# Autodesk Inventor assembly: Right Leg Assembly
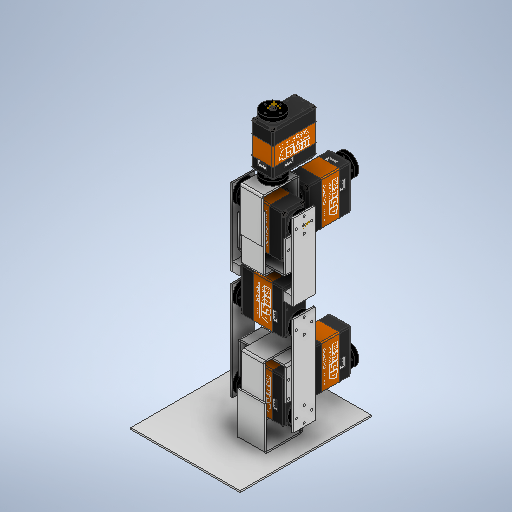
[picture p0: Inventor's stored thumbnail of the model, 512x512]
Saved by Autodesk Inventor 2025.2 (Build 292293000, 293)
## iProperties
Created: 2025-05-04
Part Number: Right Leg Assembly
Document SubType Name: Assembly
Designer: User
Author: User
## Documents named in this file (10)
- C:\Users\User\Documents\The Maverick's Files\College 3-3\로보인 프로젝트\Leg Parts\Right Leg Assembly.iam
- C:\Users\User\Documents\The Maverick's Files\College 3-3\로보인 프로젝트\Leg Parts\axis_12_bottom_frame(bottom).ipt
- C:\Users\User\Documents\The Maverick's Files\College 3-3\로보인 프로젝트\Leg Parts\axis_12_bottom_frame(top).ipt
- C:\Users\User\Documents\The Maverick's Files\College 3-3\로보인 프로젝트\RHp_hardware_example\Part\HTD-45H, Horn\HTD-45H Assembly.iam
- C:\Users\User\Documents\The Maverick's Files\College 3-3\로보인 프로젝트\Leg Parts\axis_10_11-connector_frame.ipt
- C:\Users\User\Documents\The Maverick's Files\College 3-3\로보인 프로젝트\Leg Parts\axis_9_bottom_frame.ipt
- C:\Users\User\Documents\The Maverick's Files\College 3-3\로보인 프로젝트\Leg Parts\axis_10_top_frame.ipt
- C:\Users\User\Documents\The Maverick's Files\College 3-3\로보인 프로젝트\Leg Parts\axis_8_10_connector_frame.ipt
- C:\Users\User\Documents\The Maverick's Files\College 3-3\로보인 프로젝트\Leg Parts\axis_7_top_frame.ipt
- C:\Users\User\Documents\The Maverick's Files\College 3-3\로보인 프로젝트\Leg Parts\3D_printed_part.ipt
## Components (19 placed, 9 different names)
1. axis_12_bottom_frame(bottom):1 — Mate:1, Mate:2, Mate:3, Mate:4, Mate:5, Mate:6, Mate:9, Mate:11, Mate:13
2. axis_12_bottom_frame(top):1 — Mate:4, Mate:5, Mate:6, Mate:10, Mate:12, Flush:1, Mate:14, Mate:15, Mate:16, Mate:22, Mate:25, Flush:5
3. HTD-45H Assembly:1 [sub-assembly] — Mate:12, Flush:1, Mate:13
4. HTD-45H Assembly:2 [sub-assembly] — Mate:9, Mate:10, Mate:11, Mate:20, Mate:21, Mate:23, Mate:24, Mate:26, Flush:2
5. HTD-45H Assembly:3 [sub-assembly] — Mate:27, Mate:28, Flush:2, Mate:29, Mate:30, Mate:31, Mate:32, Mate:35, Mate:37
6. HTD-45H Assembly:4 [sub-assembly] — Mate:33, Mate:34, Mate:35, Mate:36, Mate:40, Flush:9, Mate:44, Flush:10
7. HTD-45H Assembly:5 [sub-assembly] — Mate:41, Mate:42, Flush:9
8. HTD-45H Assembly:6 [sub-assembly] — Flush:5, Mate:36, Mate:37, Mate:38, Flush:6, Flush:7
9. axis_10_11-connector_frame:1 — Mate:23, Mate:24, Mate:25, Mate:27, Mate:28, Flush:4
10. axis_10_11-connector_frame:2 — Mate:20, Mate:21, Mate:22, Flush:3
11. axis_9_bottom_frame:1 — Mate:14, Mate:15, Mate:16, Mate:17, Mate:19
12. axis_10_top_frame:1 — Mate:17, Mate:19, Mate:26
13. axis_8_10_connector_frame:1 — Mate:29, Mate:30, Flush:3, Flush:11, Mate:45, Flush:12
14. axis_8_10_connector_frame:2 — Mate:31, Mate:32, Flush:4, Mate:33, Mate:34, Flush:13, Mate:46, Flush:14
15. axis_7_top_frame:1 — Mate:38, Flush:6, Flush:7, Mate:39, Flush:8
16. axis_9_bottom_frame:2 — Mate:39, Flush:8, Mate:40, Mate:41, Mate:42, Mate:43
17. axis_10_top_frame:2 — Mate:43, Mate:44, Flush:10
18. 3D_printed_part:1 — Flush:11, Mate:45, Flush:12
19. 3D_printed_part:2 — Flush:13, Mate:46, Flush:14
## Relationships (57: Mate 43, Flush 14)
- Mate:1: axis_12_bottom_frame(bottom):1
- Mate:2: axis_12_bottom_frame(bottom):1
- Mate:3: axis_12_bottom_frame(bottom):1
- Mate:4: axis_12_bottom_frame(bottom):1 ↔ axis_12_bottom_frame(top):1
- Mate:5 (-20 mm): axis_12_bottom_frame(bottom):1 ↔ axis_12_bottom_frame(top):1
- Mate:6 (-20 mm): axis_12_bottom_frame(bottom):1 ↔ axis_12_bottom_frame(top):1
- Mate:9: axis_12_bottom_frame(bottom):1 ↔ HTD-45H Assembly:2
- Mate:10 (-20 mm): axis_12_bottom_frame(top):1 ↔ HTD-45H Assembly:2
- Mate:11 (-30 mm): axis_12_bottom_frame(bottom):1 ↔ HTD-45H Assembly:2
- Mate:12: axis_12_bottom_frame(top):1 ↔ HTD-45H Assembly:1
- Flush:1: axis_12_bottom_frame(top):1 ↔ HTD-45H Assembly:1
- Mate:13 (-30 mm): axis_12_bottom_frame(bottom):1 ↔ HTD-45H Assembly:1
- Mate:14: axis_12_bottom_frame(top):1 ↔ axis_9_bottom_frame:1
- Mate:15: axis_12_bottom_frame(top):1 ↔ axis_9_bottom_frame:1
- Mate:16 (71.5 mm): axis_12_bottom_frame(top):1 ↔ axis_9_bottom_frame:1
- Mate:17: axis_9_bottom_frame:1 ↔ axis_10_top_frame:1
- Mate:19 (1.5 mm): axis_9_bottom_frame:1 ↔ axis_10_top_frame:1
- Mate:20: HTD-45H Assembly:2 ↔ axis_10_11-connector_frame:2
- Mate:21: HTD-45H Assembly:2 ↔ axis_10_11-connector_frame:2
- Mate:22 (20 mm): axis_12_bottom_frame(top):1 ↔ axis_10_11-connector_frame:2
- Mate:23: HTD-45H Assembly:2 ↔ axis_10_11-connector_frame:1
- Mate:24: HTD-45H Assembly:2 ↔ axis_10_11-connector_frame:1
- Mate:25 (20 mm): axis_12_bottom_frame(top):1 ↔ axis_10_11-connector_frame:1
- Mate:26: HTD-45H Assembly:2 ↔ axis_10_top_frame:1
- Mate:27: HTD-45H Assembly:3 ↔ axis_10_11-connector_frame:1
- Mate:28: HTD-45H Assembly:3 ↔ axis_10_11-connector_frame:1
- Flush:2 (-70 mm): HTD-45H Assembly:2 ↔ HTD-45H Assembly:3
- Mate:29 (-10 mm): HTD-45H Assembly:3 ↔ axis_8_10_connector_frame:1
- Mate:30: HTD-45H Assembly:3 ↔ axis_8_10_connector_frame:1
- Flush:3: axis_10_11-connector_frame:2 ↔ axis_8_10_connector_frame:1
- Mate:31 (-10 mm): HTD-45H Assembly:3 ↔ axis_8_10_connector_frame:2
- Mate:32: HTD-45H Assembly:3 ↔ axis_8_10_connector_frame:2
- Flush:4: axis_10_11-connector_frame:1 ↔ axis_8_10_connector_frame:2
- Mate:33: HTD-45H Assembly:4 ↔ axis_8_10_connector_frame:2
- Mate:34: HTD-45H Assembly:4 ↔ axis_8_10_connector_frame:2
- Mate:35 (80 mm): HTD-45H Assembly:3 ↔ HTD-45H Assembly:4
- Flush:5: axis_12_bottom_frame(top):1 ↔ HTD-45H Assembly:6
- Mate:36: HTD-45H Assembly:4 ↔ HTD-45H Assembly:6
- Mate:37 (80 mm): HTD-45H Assembly:3 ↔ HTD-45H Assembly:6
- Mate:38: HTD-45H Assembly:6 ↔ axis_7_top_frame:1
- Flush:6 (-18.5 mm): HTD-45H Assembly:6 ↔ axis_7_top_frame:1
- Flush:7: HTD-45H Assembly:6 ↔ axis_7_top_frame:1
- Mate:39: axis_7_top_frame:1 ↔ axis_9_bottom_frame:2
- Flush:8: axis_7_top_frame:1 ↔ axis_9_bottom_frame:2
- Mate:40 (10 mm): HTD-45H Assembly:4 ↔ axis_9_bottom_frame:2
- Mate:41: HTD-45H Assembly:5 ↔ axis_9_bottom_frame:2
- Mate:42: HTD-45H Assembly:5 ↔ axis_9_bottom_frame:2
- Flush:9: HTD-45H Assembly:4 ↔ HTD-45H Assembly:5
- Mate:43: axis_9_bottom_frame:2 ↔ axis_10_top_frame:2
- Mate:44: HTD-45H Assembly:4 ↔ axis_10_top_frame:2
- Flush:10: HTD-45H Assembly:4 ↔ axis_10_top_frame:2
- Flush:11: axis_8_10_connector_frame:1 ↔ 3D_printed_part:1
- Mate:45: axis_8_10_connector_frame:1 ↔ 3D_printed_part:1
- Flush:12: axis_8_10_connector_frame:1 ↔ 3D_printed_part:1
- Flush:13: axis_8_10_connector_frame:2 ↔ 3D_printed_part:2
- Mate:46: axis_8_10_connector_frame:2 ↔ 3D_printed_part:2
- Flush:14: axis_8_10_connector_frame:2 ↔ 3D_printed_part:2
